# Autodesk Inventor assembly: Drone V2
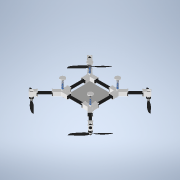
[picture p0: Inventor's stored thumbnail of the model, 180x180]
Saved by Autodesk Inventor 2022 (Build 260153000, 153)
## iProperties
Created: 2022-02-02
Part Number: Drone V2
Document SubType Name: Assembly
Designer: ultra
Author: ultra
## Documents named in this file (4)
- C:\Users\ultra\Desktop\Github\RASA-Drone\CAD Files\Drone\Drone V2.iam
- C:\Users\ultra\Desktop\Github\RASA-Drone\CAD Files\Drone\Tube.ipt
- C:\Users\ultra\Desktop\Github\RASA-Drone\CAD Files\Drone\Subframe V1.iam
- C:\Users\ultra\Desktop\Github\RASA-Drone\CAD Files\Drone\Frame.ipt
## Components (9 placed, 3 different names)
1. Tube:2 — Insert:5, Insert:9
2. Tube:10 — Insert:1, Insert:8
3. Subframe V1:1 [sub-assembly] — Insert:8, Insert:9
4. Tube:12 — Insert:3, Insert:4
5. Subframe V1:2 [sub-assembly] — Flush:1, Flush:2, Insert:1, Insert:3, Mate:1
6. Tube:13 — Insert:6, Insert:7
7. Subframe V1:3 [sub-assembly] — Insert:5, Insert:6
8. Subframe V1:4 [sub-assembly] — Flush:1, Flush:2, Insert:4, Insert:7
9. Frame:1 — Mate:1
## Relationships (11: Insert 8, Flush 2, Mate 1)
- Flush:1: Subframe V1:2 ↔ Subframe V1:4
- Flush:2: Subframe V1:2 ↔ Subframe V1:4
- Insert:1: Tube:10 ↔ Subframe V1:2
- Insert:3: Tube:12 ↔ Subframe V1:2
- Insert:4: Tube:12 ↔ Subframe V1:4
- Insert:5: Tube:2 ↔ Subframe V1:3
- Insert:6: Tube:13 ↔ Subframe V1:3
- Insert:7: Tube:13 ↔ Subframe V1:4
- Insert:8: Tube:10 ↔ Subframe V1:1
- Insert:9: Tube:2 ↔ Subframe V1:1
- Mate:1: Subframe V1:2 ↔ Frame:1
